# Autodesk Inventor assembly: GyroCopter
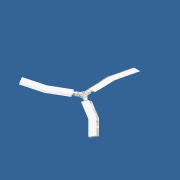
[picture p0: Inventor's stored thumbnail of the model, 180x180]
Saved by Autodesk Inventor 2022 (Build 260153000, 153)
## iProperties
Created: 2021-12-01
Part Number: GyroCopter
Document SubType Name: Assembly
Designer: Vedic
Author: Vedic
## Documents named in this file (3)
- C:\Users\Wilson\OneDrive\Documents\Projekts\Rocketery\CAD Files v1\Rocoverey System Gyro\Aerospace\GyroCopter.iam
- C:\Users\Wilson\OneDrive\Documents\Projekts\Rocketery\CAD Files v1\Rocoverey System Gyro\Aerospace\Gyrocopter Base.ipt
- C:\Users\Wilson\OneDrive\Documents\Projekts\Rocketery\CAD Files v1\Rocoverey System Gyro\Aerospace\Gyrocopter Blade.ipt
## Components (4 placed, 2 different names)
1. Gyrocopter Blade:1 — Mate:3, Mate:6
2. Gyrocopter Blade:2 — Mate:1, Mate:2
3. Gyrocopter Blade:3 — Mate:4, Mate:5
4. Gyrocopter Base:1 — Mate:1, Mate:2, Mate:3, Mate:4, Mate:5, Mate:6
## Relationships (6: Mate 6)
- Mate:1: Gyrocopter Blade:2 ↔ Gyrocopter Base:1
- Mate:2: Gyrocopter Blade:2 ↔ Gyrocopter Base:1
- Mate:3: Gyrocopter Blade:1 ↔ Gyrocopter Base:1
- Mate:4: Gyrocopter Blade:3 ↔ Gyrocopter Base:1
- Mate:5: Gyrocopter Blade:3 ↔ Gyrocopter Base:1
- Mate:6: Gyrocopter Blade:1 ↔ Gyrocopter Base:1
